# Autodesk Inventor assembly: Ensemble1
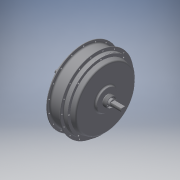
[picture p0: Inventor's stored thumbnail of the model, 180x180]
Saved by Autodesk Inventor 2016 (Build 200138000, 138)
## iProperties
Created: 2015-11-15
Part Number: Ensemble1
Material: Générique
Document SubType Name: Assembly
Designer: Cyril
Author: Cyril
## Documents named in this file (5)
- C:\Users\Yann\Documents\GitHub\Bikair_CAD\Source\Rear_Train\Motor\Motor.iam
- C:\Users\Yann\Documents\GitHub\Bikair_CAD\Source\Rear_Train\Motor\Rotor_Rim.ipt
- C:\Users\Yann\Documents\GitHub\Bikair_CAD\Source\Rear_Train\Motor\Rotor_Left_Cover.ipt
- C:\Users\Yann\Documents\GitHub\Bikair_CAD\Source\Rear_Train\Motor\Rotor_Right_Cover.ipt
- C:\Users\Yann\Documents\GitHub\Bikair_CAD\Source\Rear_Train\Motor\Stator_Axis.ipt
## Components (4 placed, 4 different names)
1. Stator_Axis:1 — Affleurement:1, Affleurement:2, Affleurement:3, Logement:1, Logement:2
2. Rotor_Rim:1 — Logement:3, Logement:4, Logement:5
3. Rotor_Left_Cover:1 — Logement:1, Logement:3, Logement:4, Placage:1
4. Rotor_Right_Cover:1 — Logement:2, Logement:5
## Relationships (9: Insert 5, Flush 3, Mate 1)
- Affleurement:1 [Flush]: Stator_Axis:1
- Affleurement:2 [Flush]: Stator_Axis:1
- Affleurement:3 [Flush]: Stator_Axis:1
- Logement:1 [Insert] (32 mm): Stator_Axis:1 ↔ Rotor_Left_Cover:1
- Logement:2 [Insert] (23.5 mm): Stator_Axis:1 ↔ Rotor_Right_Cover:1
- Logement:3 [Insert]: Rotor_Rim:1 ↔ Rotor_Left_Cover:1
- Logement:4 [Insert]: Rotor_Rim:1 ↔ Rotor_Left_Cover:1
- Logement:5 [Insert]: Rotor_Rim:1 ↔ Rotor_Right_Cover:1
- Placage:1 [Mate]: Rotor_Left_Cover:1
